# Autodesk Inventor assembly: Chest Assembly
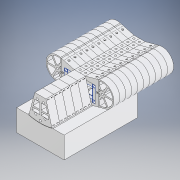
[picture p0: Inventor's stored thumbnail of the model, 180x180]
Saved by Autodesk Inventor 2017 SP1 (Build 210196100, 196)
## iProperties
Created: 2017-06-04
Part Number: Chest Assembly
Document SubType Name: Assembly
Designer: Zach
Author: Zach
## Documents named in this file (5)
- C:\Users\Zach\Documents\GitHub\tr1\src\Body\Chest Assembly\Chest Assembly.iam
- C:\Users\Zach\Documents\GitHub\tr1\src\Body\Chest Assembly\CA001.ipt
- C:\Users\Zach\Documents\GitHub\tr1\src\Body\Chest Assembly\CA002.ipt
- C:\Users\Zach\Documents\GitHub\tr1\src\Body\Chest Assembly\Rise Base Assembly\Riser Base.iam
- C:\Users\Zach\Documents\GitHub\tr1\src\Body\Chest Assembly\Chassis\Chassis.iam
## Components (8 placed, 4 different names)
1. CA001:1 — Flush:1, Flush:2, Flush:3, Flush:4, Flush:5, Flush:6, Flush:7, Flush:8, Mate:1, Mate:15, Mate:18, Mate:19, Mate:21
2. CA001:2 — Flush:2, Flush:8, Mate:1, Mate:2
3. CA001:3 — Flush:3, Flush:7, Mate:4, Flush:9, Mate:20
4. CA001:4 — Flush:4, Flush:6, Mate:2, Mate:3
5. CA001:5 — Flush:1, Flush:5, Mate:3, Mate:4
6. CA002:1 — Flush:9, Mate:20, Mate:21
7. Riser Base:1 [sub-assembly] — Mate:15, Mate:16, Mate:17, Mate:18, Mate:19
8. Chassis:1 [sub-assembly] — Mate:16, Mate:17
## Relationships (20: Mate 11, Flush 9)
- Flush:1: CA001:1 ↔ CA001:5
- Flush:2: CA001:1 ↔ CA001:2
- Flush:3: CA001:1 ↔ CA001:3
- Flush:4: CA001:1 ↔ CA001:4
- Flush:5: CA001:1 ↔ CA001:5
- Flush:6: CA001:1 ↔ CA001:4
- Flush:7: CA001:1 ↔ CA001:3
- Flush:8: CA001:1 ↔ CA001:2
- Mate:1: CA001:1 ↔ CA001:2
- Mate:2: CA001:2 ↔ CA001:4
- Mate:3: CA001:4 ↔ CA001:5
- Mate:4: CA001:3 ↔ CA001:5
- Flush:9: CA001:3 ↔ CA002:1
- Mate:15: CA001:1 ↔ Riser Base:1
- Mate:16: Riser Base:1 ↔ Chassis:1
- Mate:17: Riser Base:1 ↔ Chassis:1
- Mate:18: CA001:1 ↔ Riser Base:1
- Mate:19: CA001:1 ↔ Riser Base:1
- Mate:20: CA001:3 ↔ CA002:1
- Mate:21: CA001:1 ↔ CA002:1
